# Autodesk Inventor assembly: Protocube
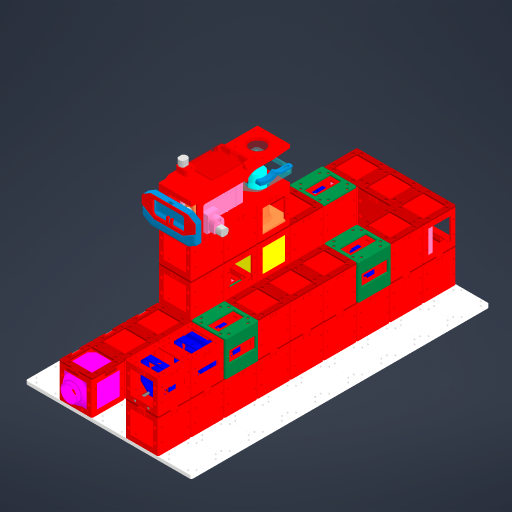
[picture p0: Inventor's stored thumbnail of the model, 512x512]
Saved by Autodesk Inventor 2023.4 (Build 274418000, 418)
## iProperties
Created: 2022-08-13
Part Number: Protocube
Document SubType Name: Assembly
Designer: xSibe
Author: xSibe
## Documents named in this file (20)
- C:\.Laptop\.Work\Projects\Project Protocube\Protocube\CAD, STL, OBJ Files\1 CAD\Protocube.iam
- C:\.Laptop\.Work\Projects\Project Protocube\Protocube\CAD, STL, OBJ Files\1 CAD\Baseplates\Baseplate 9x5 V5.ipt
- C:\.Laptop\.Work\Projects\Project Protocube\Protocube\CAD, STL, OBJ Files\1 CAD\Lens\Cube 1x1 V5 (Half Inch Lens).iam
- C:\.Laptop\.Work\Projects\Project Protocube\Protocube\CAD, STL, OBJ Files\1 CAD\Mirror\Cube 1x1 V5 (Mirror Horizontal).iam
- C:\.Laptop\.Work\Projects\Project Protocube\Protocube\CAD, STL, OBJ Files\1 CAD\Cubes\Cube 1x1 V5 Closed Horizontal.iam
- C:\.Laptop\.Work\Projects\Project Protocube\Protocube\CAD, STL, OBJ Files\1 CAD\Lens\Cube 1x1 V5 (One Inch Lens).iam
- C:\.Laptop\.Work\Projects\Project Protocube\Protocube\CAD, STL, OBJ Files\1 CAD\XYZ Stage\XYZ Stage V5.iam
- C:\.Laptop\.Work\Projects\Project Protocube\Protocube\CAD, STL, OBJ Files\1 CAD\Mirror\Cube 1x1 V5 (Mirror Vertical).iam
- C:\.Laptop\.Work\Projects\Project Protocube\Protocube\CAD, STL, OBJ Files\1 CAD\Laser\Cube 1x1 V5 (USB Laser).iam
- C:\.Laptop\.Work\Projects\Project Protocube\Protocube\CAD, STL, OBJ Files\1 CAD\Camera\Cube 1x1 V5 (Camera).iam
- C:\.Laptop\.Work\Projects\Project Protocube\Protocube\CAD, STL, OBJ Files\1 CAD\Dichroic\Cube 1x1 V5 (Dichroic).iam
- C:\.Laptop\.Work\Projects\Project Protocube\Protocube\CAD, STL, OBJ Files\1 CAD\Objective\Cube 1x1 V5 (Objective).iam
- C:\.Laptop\.Work\Projects\Project Protocube\Protocube\CAD, STL, OBJ Files\1 CAD\Gamepad\Gamepad Enclosure.iam
- C:\.Laptop\.Work\Projects\Project Protocube\Protocube\CAD, STL, OBJ Files\1 CAD\Sample\Cube (Sample).iam
- C:\.Laptop\.Work\Projects\Project Protocube\Protocube\CAD, STL, OBJ Files\1 CAD\Baseplates\Interlinking Baseplate.ipt
- C:\.Laptop\.Work\Projects\Project Protocube\Protocube\CAD, STL, OBJ Files\1 CAD\Baseplates\Interlinking Baseplate Pathed Male.ipt
- C:\.Laptop\.Work\Projects\Project Protocube\Protocube\CAD, STL, OBJ Files\1 CAD\Baseplates\Interlinking Baseplate Pathed Female.ipt
- C:\.Laptop\.Work\Projects\Project Protocube\Protocube\CAD, STL, OBJ Files\1 CAD\Baseplates\Interlinking Baseplate Pathed.ipt
- C:\.Laptop\.Work\Projects\Project Protocube\Protocube\CAD, STL, OBJ Files\1 CAD\Baseplates\Interlinking Baseplate Pathed Angle V2.ipt
- C:\.Laptop\.Work\Projects\Project Protocube\Protocube\CAD, STL, OBJ Files\1 CAD\Cubes\Cube 1x1 V5.iam
## Components (70 placed, 19 different names)
1. Baseplate 9x5 V5:1 — Mate:60, Mate:61, Mate:62, Mate:65, Mate:66, Mate:67, Mate:69, Mate:70, Mate:71, Mate:93, Mate:94, Mate:95, Mate:98, Mate:99, Mate:100, Mate:101, Mate:102, Mate:103, Mate:107, Mate:108, Mate:109, Mate:118, Mate:119, Mate:120
2. Cube 1x1 V5 (Mirror Horizontal):1 [sub-assembly] — Mate:81, Flush:14, Flush:15, Mate:157, Mate:158, Mate:159
3. Cube 1x1 V5 (Mirror Horizontal):2 [sub-assembly] — Flush:16, Flush:17, Mate:82, Mate:151, Mate:152, Mate:153
4. Cube 1x1 V5 (Half Inch Lens):1 [sub-assembly] — Mate:77, Flush:8, Flush:9
5. Cube 1x1 V5 (One Inch Lens):1 [sub-assembly] — Mate:96, Flush:87, Flush:88
6. Cube 1x1 V5 (One Inch Lens):2 [sub-assembly] — Mate:97, Flush:89, Flush:90
7. Cube 1x1 V5 (One Inch Lens):3 [sub-assembly] — Mate:98, Mate:99, Mate:100, Mate:175, Mate:176, Mate:177
8. Cube 1x1 V5 (Mirror Vertical):1 [sub-assembly] — Mate:101, Mate:102, Mate:103, Mate:110, Flush:91, Flush:92
9. Cube 1x1 V5 (USB Laser):1 [sub-assembly] — Mate:104, Mate:105, Mate:106
10. Cube 1x1 V5 (Camera):1 [sub-assembly] — Mate:107, Mate:108, Mate:109, Mate:172, Mate:173, Mate:174
11. Cube 1x1 V5 (Dichroic):1 [sub-assembly] — Mate:110, Flush:91, Flush:92, Mate:111, Flush:93, Flush:94, Mate:145, Mate:147, Mate:148
12. Cube 1x1 V5 (Objective):1 [sub-assembly] — Mate:111, Flush:93, Flush:94, Mate:113, Mate:114, Mate:115
13. Gamepad Enclosure:1 [sub-assembly] — Mate:112, Mate:116, Mate:117
14. Cube (Sample):1 [sub-assembly] — Mate:118, Mate:119, Mate:120
15. XYZ Stage V5:1 [sub-assembly] — Mate:112, Mate:113, Mate:114, Mate:115, Mate:116, Mate:117
16. Cube 1x1 V5:1 [sub-assembly] — Mate:175, Mate:176, Mate:177
17. Cube 1x1 V5 Closed Horizontal:27 [sub-assembly] — Mate:178, Mate:179, Mate:180
18. Interlinking Baseplate:10 — Mate:124, Mate:125, Mate:126
19. Interlinking Baseplate Pathed:3 — Mate:154, Mate:155, Mate:156
20. Interlinking Baseplate Pathed:4 — Mate:166, Mate:167, Mate:168
21. Interlinking Baseplate Pathed Male:1 — Mate:142, Mate:143, Mate:144
22. Interlinking Baseplate Pathed Male:2 — Mate:151, Mate:152, Mate:153
23. Interlinking Baseplate Pathed Male:3 — Mate:163, Mate:164, Mate:165
24. Interlinking Baseplate Pathed Female:1 — Mate:146, Mate:149, Mate:150
25. Interlinking Baseplate Pathed Female:2 — Mate:160, Mate:161, Mate:162
26. Interlinking Baseplate Pathed Female:3 — Mate:169, Mate:170, Mate:171
27. Interlinking Baseplate Pathed Angle V2:1 — Mate:157, Mate:158, Mate:159
28. Cube 1x1 V5 Closed Horizontal:13 [sub-assembly] — Flush:3, Mate:80, Flush:13, Mate:160, Mate:161, Mate:162
29. Cube 1x1 V5 Closed Horizontal:17 [sub-assembly] — Flush:20, Flush:21, Mate:84, Mate:142, Mate:143, Mate:144
30. Interlinking Baseplate:1 — Mate:121, Mate:122, Mate:123
31. Interlinking Baseplate:2
32. Interlinking Baseplate:3
33. Interlinking Baseplate:4
34. Interlinking Baseplate:5
35. Interlinking Baseplate:6
36. Interlinking Baseplate:7
37. Interlinking Baseplate:8
38. Interlinking Baseplate:9
39. Interlinking Baseplate:11 — Mate:127, Mate:128, Mate:129
40. Interlinking Baseplate:12
41. Interlinking Baseplate:13
42. Interlinking Baseplate:14
43. Interlinking Baseplate Pathed:1 — Mate:145, Mate:147, Mate:148
44. Interlinking Baseplate Pathed:2 — Mate:178, Mate:179, Mate:180
45. Interlinking Baseplate:15 — Mate:172, Mate:173, Mate:174
46. Interlinking Baseplate:16
47. Interlinking Baseplate:17
48. Interlinking Baseplate:18
49. Cube 1x1 V5 Closed Horizontal:1 [sub-assembly] — Mate:60, Mate:61, Mate:62, Mate:104, Mate:105, Mate:106, Mate:121, Mate:122, Mate:123
50. Cube 1x1 V5 Closed Horizontal:2 [sub-assembly]
51. Cube 1x1 V5 Closed Horizontal:3 [sub-assembly] — Mate:77, Flush:8, Flush:9
52. Cube 1x1 V5 Closed Horizontal:4 [sub-assembly] — Flush:2, Mate:78, Flush:10
53. Cube 1x1 V5 Closed Horizontal:5 [sub-assembly]
54. Cube 1x1 V5 Closed Horizontal:6 [sub-assembly]
55. Cube 1x1 V5 Closed Horizontal:7 [sub-assembly] — Mate:96, Flush:87, Flush:88
56. Cube 1x1 V5 Closed Horizontal:8 [sub-assembly] — Flush:3, Mate:80, Flush:13
57. Cube 1x1 V5 Closed Horizontal:9 [sub-assembly] — Mate:81, Flush:14, Flush:15
58. Cube 1x1 V5 Closed Horizontal:10 [sub-assembly] — Flush:2, Mate:78, Flush:10, Mate:163, Mate:164, Mate:165
59. Cube 1x1 V5 Closed Horizontal:11 [sub-assembly] — Mate:166, Mate:167, Mate:168
60. Cube 1x1 V5 Closed Horizontal:12 [sub-assembly] — Mate:169, Mate:170, Mate:171
61. Cube 1x1 V5 Closed Horizontal:14 [sub-assembly] — Mate:65, Mate:66, Mate:67, Flush:16, Flush:17, Mate:82, Mate:127, Mate:128, Mate:129
62. Cube 1x1 V5 Closed Horizontal:15 [sub-assembly] — Mate:97, Flush:89, Flush:90
63. Cube 1x1 V5 Closed Horizontal:16 [sub-assembly] — Flush:20, Mate:84, Flush:21
64. Cube 1x1 V5 Closed Horizontal:18 [sub-assembly] — Mate:69, Mate:70, Mate:71, Flush:5, Mate:91, Flush:27
65. Cube 1x1 V5 Closed Horizontal:19 [sub-assembly]
66. Cube 1x1 V5 Closed Horizontal:20 [sub-assembly]
67. Cube 1x1 V5 Closed Horizontal:21 [sub-assembly] — Flush:5, Mate:91, Flush:27, Mate:146, Mate:149, Mate:150
68. Cube 1x1 V5 Closed Horizontal:22 [sub-assembly]
69. Cube 1x1 V5 Closed Horizontal:25 [sub-assembly] — Mate:93, Mate:94, Mate:95, Mate:124, Mate:125, Mate:126
70. Cube 1x1 V5 Closed Horizontal:26 [sub-assembly] — Mate:154, Mate:155, Mate:156
## Component patterns: (9 elements, first: Interlinking Baseplate:1), (4 elements, first: Interlinking Baseplate:11), (2 elements, first: Interlinking Baseplate Pathed:1), (4 elements, first: Interlinking Baseplate:15), (9 elements, first: Cube 1x1 V5 Closed Horizontal:1), (3 elements, first: Cube 1x1 V5 Closed Horizontal:10), (3 elements, first: Cube 1x1 V5 Closed Horizontal:14), (3 elements, first: Cube 1x1 V5 Closed Horizontal:18), (2 elements, first: Cube 1x1 V5 Closed Horizontal:21), (2 elements, first: Cube 1x1 V5 Closed Horizontal:25)
## Relationships (114: Mate 92, Flush 22)
- Mate:60: Baseplate 9x5 V5:1 ↔ Cube 1x1 V5 Closed Horizontal:1
- Mate:61: Baseplate 9x5 V5:1 ↔ Cube 1x1 V5 Closed Horizontal:1
- Mate:62: Baseplate 9x5 V5:1 ↔ Cube 1x1 V5 Closed Horizontal:1
- Flush:2: Cube 1x1 V5 Closed Horizontal:4 ↔ Cube 1x1 V5 Closed Horizontal:10
- Flush:3: Cube 1x1 V5 Closed Horizontal:13 ↔ Cube 1x1 V5 Closed Horizontal:8
- Mate:65: Baseplate 9x5 V5:1 ↔ Cube 1x1 V5 Closed Horizontal:14
- Mate:66: Baseplate 9x5 V5:1 ↔ Cube 1x1 V5 Closed Horizontal:14
- Mate:67: Baseplate 9x5 V5:1 ↔ Cube 1x1 V5 Closed Horizontal:14
- Mate:69: Baseplate 9x5 V5:1 ↔ Cube 1x1 V5 Closed Horizontal:18
- Mate:70: Baseplate 9x5 V5:1 ↔ Cube 1x1 V5 Closed Horizontal:18
- Mate:71: Baseplate 9x5 V5:1 ↔ Cube 1x1 V5 Closed Horizontal:18
- Flush:5: Cube 1x1 V5 Closed Horizontal:18 ↔ Cube 1x1 V5 Closed Horizontal:21
- Mate:77 (2 mm): Cube 1x1 V5 (Half Inch Lens):1 ↔ Cube 1x1 V5 Closed Horizontal:3
- Flush:8: Cube 1x1 V5 (Half Inch Lens):1 ↔ Cube 1x1 V5 Closed Horizontal:3
- Flush:9: Cube 1x1 V5 (Half Inch Lens):1 ↔ Cube 1x1 V5 Closed Horizontal:3
- Mate:78 (2 mm): Cube 1x1 V5 Closed Horizontal:4 ↔ Cube 1x1 V5 Closed Horizontal:10
- Flush:10: Cube 1x1 V5 Closed Horizontal:4 ↔ Cube 1x1 V5 Closed Horizontal:10
- Mate:80 (2 mm): Cube 1x1 V5 Closed Horizontal:13 ↔ Cube 1x1 V5 Closed Horizontal:8
- Flush:13: Cube 1x1 V5 Closed Horizontal:13 ↔ Cube 1x1 V5 Closed Horizontal:8
- Mate:81 (2 mm): Cube 1x1 V5 (Mirror Horizontal):1 ↔ Cube 1x1 V5 Closed Horizontal:9
- Flush:14: Cube 1x1 V5 (Mirror Horizontal):1 ↔ Cube 1x1 V5 Closed Horizontal:9
- Flush:15: Cube 1x1 V5 (Mirror Horizontal):1 ↔ Cube 1x1 V5 Closed Horizontal:9
- Flush:16: Cube 1x1 V5 (Mirror Horizontal):2 ↔ Cube 1x1 V5 Closed Horizontal:14
- Flush:17: Cube 1x1 V5 (Mirror Horizontal):2 ↔ Cube 1x1 V5 Closed Horizontal:14
- Mate:82 (2 mm): Cube 1x1 V5 (Mirror Horizontal):2 ↔ Cube 1x1 V5 Closed Horizontal:14
- Flush:20: Cube 1x1 V5 Closed Horizontal:17 ↔ Cube 1x1 V5 Closed Horizontal:16
- Flush:21: Cube 1x1 V5 Closed Horizontal:17 ↔ Cube 1x1 V5 Closed Horizontal:16
- Mate:84 (2 mm): Cube 1x1 V5 Closed Horizontal:17 ↔ Cube 1x1 V5 Closed Horizontal:16
- Mate:91 (2 mm): Cube 1x1 V5 Closed Horizontal:18 ↔ Cube 1x1 V5 Closed Horizontal:21
- Flush:27: Cube 1x1 V5 Closed Horizontal:18 ↔ Cube 1x1 V5 Closed Horizontal:21
- Mate:93: Baseplate 9x5 V5:1 ↔ Cube 1x1 V5 Closed Horizontal:25
- Mate:94: Baseplate 9x5 V5:1 ↔ Cube 1x1 V5 Closed Horizontal:25
- Mate:95: Baseplate 9x5 V5:1 ↔ Cube 1x1 V5 Closed Horizontal:25
- Mate:96 (2 mm): Cube 1x1 V5 (One Inch Lens):1 ↔ Cube 1x1 V5 Closed Horizontal:7
- Flush:87: Cube 1x1 V5 (One Inch Lens):1 ↔ Cube 1x1 V5 Closed Horizontal:7
- Flush:88: Cube 1x1 V5 (One Inch Lens):1 ↔ Cube 1x1 V5 Closed Horizontal:7
- Mate:97 (2 mm): Cube 1x1 V5 (One Inch Lens):2 ↔ Cube 1x1 V5 Closed Horizontal:15
- Flush:89: Cube 1x1 V5 (One Inch Lens):2 ↔ Cube 1x1 V5 Closed Horizontal:15
- Flush:90: Cube 1x1 V5 (One Inch Lens):2 ↔ Cube 1x1 V5 Closed Horizontal:15
- Mate:98: Baseplate 9x5 V5:1 ↔ Cube 1x1 V5 (One Inch Lens):3
- Mate:99: Baseplate 9x5 V5:1 ↔ Cube 1x1 V5 (One Inch Lens):3
- Mate:100: Baseplate 9x5 V5:1 ↔ Cube 1x1 V5 (One Inch Lens):3
- Mate:101: Baseplate 9x5 V5:1 ↔ Cube 1x1 V5 (Mirror Vertical):1
- Mate:102: Baseplate 9x5 V5:1 ↔ Cube 1x1 V5 (Mirror Vertical):1
- Mate:103: Baseplate 9x5 V5:1 ↔ Cube 1x1 V5 (Mirror Vertical):1
- Mate:104 (2 mm): Cube 1x1 V5 (USB Laser):1 ↔ Cube 1x1 V5 Closed Horizontal:1
- Mate:105: Cube 1x1 V5 (USB Laser):1 ↔ Cube 1x1 V5 Closed Horizontal:1
- Mate:106: Cube 1x1 V5 (USB Laser):1 ↔ Cube 1x1 V5 Closed Horizontal:1
- Mate:107: Baseplate 9x5 V5:1 ↔ Cube 1x1 V5 (Camera):1
- Mate:108: Baseplate 9x5 V5:1 ↔ Cube 1x1 V5 (Camera):1
- Mate:109: Baseplate 9x5 V5:1 ↔ Cube 1x1 V5 (Camera):1
- Mate:110 (2 mm): Cube 1x1 V5 (Mirror Vertical):1 ↔ Cube 1x1 V5 (Dichroic):1
- Flush:91: Cube 1x1 V5 (Mirror Vertical):1 ↔ Cube 1x1 V5 (Dichroic):1
- Flush:92: Cube 1x1 V5 (Mirror Vertical):1 ↔ Cube 1x1 V5 (Dichroic):1
- Mate:111 (2 mm): Cube 1x1 V5 (Dichroic):1 ↔ Cube 1x1 V5 (Objective):1
- Flush:93: Cube 1x1 V5 (Dichroic):1 ↔ Cube 1x1 V5 (Objective):1
- Flush:94: Cube 1x1 V5 (Dichroic):1 ↔ Cube 1x1 V5 (Objective):1
- Mate:112: Gamepad Enclosure:1 ↔ XYZ Stage V5:1
- Mate:113: Cube 1x1 V5 (Objective):1 ↔ XYZ Stage V5:1
- Mate:114: Cube 1x1 V5 (Objective):1 ↔ XYZ Stage V5:1
- Mate:115: Cube 1x1 V5 (Objective):1 ↔ XYZ Stage V5:1
- Mate:116: Gamepad Enclosure:1 ↔ XYZ Stage V5:1
- Mate:117: Gamepad Enclosure:1 ↔ XYZ Stage V5:1
- Mate:118: Baseplate 9x5 V5:1 ↔ Cube (Sample):1
- Mate:119: Baseplate 9x5 V5:1 ↔ Cube (Sample):1
- Mate:120: Baseplate 9x5 V5:1 ↔ Cube (Sample):1
- Mate:121: Interlinking Baseplate:1 ↔ Cube 1x1 V5 Closed Horizontal:1
- Mate:122: Interlinking Baseplate:1 ↔ Cube 1x1 V5 Closed Horizontal:1
- Mate:123: Interlinking Baseplate:1 ↔ Cube 1x1 V5 Closed Horizontal:1
- Mate:124: Interlinking Baseplate:10 ↔ Cube 1x1 V5 Closed Horizontal:25
- Mate:125: Interlinking Baseplate:10 ↔ Cube 1x1 V5 Closed Horizontal:25
- Mate:126: Interlinking Baseplate:10 ↔ Cube 1x1 V5 Closed Horizontal:25
- Mate:127: Interlinking Baseplate:11 ↔ Cube 1x1 V5 Closed Horizontal:14
- Mate:128: Interlinking Baseplate:11 ↔ Cube 1x1 V5 Closed Horizontal:14
- Mate:129: Interlinking Baseplate:11 ↔ Cube 1x1 V5 Closed Horizontal:14
- Mate:142: Interlinking Baseplate Pathed Male:1 ↔ Cube 1x1 V5 Closed Horizontal:17
- Mate:143: Interlinking Baseplate Pathed Male:1 ↔ Cube 1x1 V5 Closed Horizontal:17
- Mate:144: Interlinking Baseplate Pathed Male:1 ↔ Cube 1x1 V5 Closed Horizontal:17
- Mate:145: Cube 1x1 V5 (Dichroic):1 ↔ Interlinking Baseplate Pathed:1
- Mate:146: Interlinking Baseplate Pathed Female:1 ↔ Cube 1x1 V5 Closed Horizontal:21
- Mate:147: Cube 1x1 V5 (Dichroic):1 ↔ Interlinking Baseplate Pathed:1
- Mate:148: Cube 1x1 V5 (Dichroic):1 ↔ Interlinking Baseplate Pathed:1
- Mate:149: Interlinking Baseplate Pathed Female:1 ↔ Cube 1x1 V5 Closed Horizontal:21
- Mate:150: Interlinking Baseplate Pathed Female:1 ↔ Cube 1x1 V5 Closed Horizontal:21
- Mate:151: Cube 1x1 V5 (Mirror Horizontal):2 ↔ Interlinking Baseplate Pathed Male:2
- Mate:152: Cube 1x1 V5 (Mirror Horizontal):2 ↔ Interlinking Baseplate Pathed Male:2
- Mate:153: Cube 1x1 V5 (Mirror Horizontal):2 ↔ Interlinking Baseplate Pathed Male:2
- Mate:154: Interlinking Baseplate Pathed:3 ↔ Cube 1x1 V5 Closed Horizontal:26
- Mate:155: Interlinking Baseplate Pathed:3 ↔ Cube 1x1 V5 Closed Horizontal:26
- Mate:156: Interlinking Baseplate Pathed:3 ↔ Cube 1x1 V5 Closed Horizontal:26
- Mate:157: Cube 1x1 V5 (Mirror Horizontal):1 ↔ Interlinking Baseplate Pathed Angle V2:1
- Mate:158: Cube 1x1 V5 (Mirror Horizontal):1 ↔ Interlinking Baseplate Pathed Angle V2:1
- Mate:159: Cube 1x1 V5 (Mirror Horizontal):1 ↔ Interlinking Baseplate Pathed Angle V2:1
- Mate:160: Interlinking Baseplate Pathed Female:2 ↔ Cube 1x1 V5 Closed Horizontal:13
- Mate:161: Interlinking Baseplate Pathed Female:2 ↔ Cube 1x1 V5 Closed Horizontal:13
- Mate:162: Interlinking Baseplate Pathed Female:2 ↔ Cube 1x1 V5 Closed Horizontal:13
- Mate:163: Interlinking Baseplate Pathed Male:3 ↔ Cube 1x1 V5 Closed Horizontal:10
- Mate:164: Interlinking Baseplate Pathed Male:3 ↔ Cube 1x1 V5 Closed Horizontal:10
- Mate:165: Interlinking Baseplate Pathed Male:3 ↔ Cube 1x1 V5 Closed Horizontal:10
- Mate:166: Interlinking Baseplate Pathed:4 ↔ Cube 1x1 V5 Closed Horizontal:11
- Mate:167: Interlinking Baseplate Pathed:4 ↔ Cube 1x1 V5 Closed Horizontal:11
- Mate:168: Interlinking Baseplate Pathed:4 ↔ Cube 1x1 V5 Closed Horizontal:11
- Mate:169: Interlinking Baseplate Pathed Female:3 ↔ Cube 1x1 V5 Closed Horizontal:12
- Mate:170: Interlinking Baseplate Pathed Female:3 ↔ Cube 1x1 V5 Closed Horizontal:12
- Mate:171: Interlinking Baseplate Pathed Female:3 ↔ Cube 1x1 V5 Closed Horizontal:12
- Mate:172: Cube 1x1 V5 (Camera):1 ↔ Interlinking Baseplate:15
- Mate:173: Cube 1x1 V5 (Camera):1 ↔ Interlinking Baseplate:15
- Mate:174: Cube 1x1 V5 (Camera):1 ↔ Interlinking Baseplate:15
- Mate:175: Cube 1x1 V5 (One Inch Lens):3 ↔ Cube 1x1 V5:1
- Mate:176: Cube 1x1 V5 (One Inch Lens):3 ↔ Cube 1x1 V5:1
- Mate:177: Cube 1x1 V5 (One Inch Lens):3 ↔ Cube 1x1 V5:1
- Mate:178: Cube 1x1 V5 Closed Horizontal:27 ↔ Interlinking Baseplate Pathed:2
- Mate:179: Cube 1x1 V5 Closed Horizontal:27 ↔ Interlinking Baseplate Pathed:2
- Mate:180: Cube 1x1 V5 Closed Horizontal:27 ↔ Interlinking Baseplate Pathed:2
